# Autodesk Inventor assembly: Motor+ArmToArm
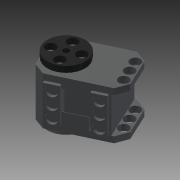
[picture p0: Inventor's stored thumbnail of the model, 180x180]
Saved by Autodesk Inventor 2014 (Build 180170000, 170)
## iProperties
Created: 2014-03-07
Part Number: Motor+ArmToArm
Document SubType Name: Assembly
Designer: Grégoire
Author: Grégoire
## Documents named in this file (4)
- C:\Users\Bless\Desktop\XL320\src\Motor+ArmToArm.iam
- C:\Users\Bless\Desktop\XL320\src\Motor.ipt
- C:\Users\Bless\Desktop\XL320\src\Arm.ipt
- C:\Users\Bless\Desktop\XL320\src\CounterArm.ipt
## Components (3 placed, 3 different names)
1. Motor:1 — Placage:1, Placage:2, Placage:3, Placage:4
2. Arm:1 — Placage:3, Placage:4
3. CounterArm:1 — Placage:1, Placage:2
## Relationships (4: Mate 4)
- Placage:1 [Mate]: Motor:1 ↔ CounterArm:1
- Placage:2 [Mate]: Motor:1 ↔ CounterArm:1
- Placage:3 [Mate]: Motor:1 ↔ Arm:1
- Placage:4 [Mate]: Motor:1 ↔ Arm:1
